# Autodesk Inventor assembly: 3.25'' Traction Wheel, Square Insert2
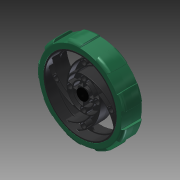
[picture p0: Inventor's stored thumbnail of the model, 180x180]
Saved by Autodesk Inventor 2015 SP1 (Build 190201100, 201)
## iProperties
Company: Bots 'n' Stuff
Created: 2014-08-29
Document SubType Name: Assembly
Designer: Jordan Kiesel
Vendor: VEX Robotics, Inc.
Mass: 57.114 g
Surface Area: 417.458 cm^2
Volume: 47.1689 cm^3
Density: 1.21084 g/cm^3
Part Number: 3.25'' Traction Wheel, Square Insert2
Author: Jordan Kiesel
Title: 3.25" Traction Wheel, Square Insert
## Documents named in this file (3)
- C:\Users\Jordan\Documents\Robotics\VEX\CAD\2015 BNS CAD Library (beta)\Motion\Wheels & Rollers\3.25'' Traction Wheel, Square Insert2.iam
- C:\Users\Jordan\Documents\Robotics\VEX\CAD\2015 BNS CAD Library (beta)\Motion\Wheels & Rollers\Reference Parts\3.25'' Traction Wheels\3.25'' Traction Wheel.iam
- C:\Users\Jordan\Documents\Robotics\VEX\CAD\2015 BNS CAD Library (beta)\Motion\Reference Parts\High Strength Square Gear Insert.ipt
## Components (3 placed, 2 different names)
1. 3.25'' Traction Wheel:1 [sub-assembly] — Mate:1, Mate:2, Mate:3, Mate:4, Mate:5, Mate:6
2. High Strength Square Gear Insert:1 — Mate:1, Mate:2, Mate:3
3. High Strength Square Gear Insert:2 — Mate:4, Mate:5, Mate:6
## Relationships (6: Mate 6)
- Mate:1 (0.0254 mm): 3.25'' Traction Wheel:1 ↔ High Strength Square Gear Insert:1
- Mate:2 (0.0254 mm): 3.25'' Traction Wheel:1 ↔ High Strength Square Gear Insert:1
- Mate:3: 3.25'' Traction Wheel:1 ↔ High Strength Square Gear Insert:1
- Mate:4 (0.0254 mm): 3.25'' Traction Wheel:1 ↔ High Strength Square Gear Insert:2
- Mate:5 (0.0254 mm): 3.25'' Traction Wheel:1 ↔ High Strength Square Gear Insert:2
- Mate:6: 3.25'' Traction Wheel:1 ↔ High Strength Square Gear Insert:2
